# Autodesk Inventor assembly: WheelAssembly3.0
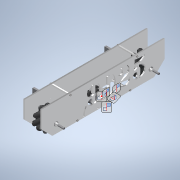
[picture p0: Inventor's stored thumbnail of the model, 180x180]
Saved by Autodesk Inventor 2021 (Build 250183000, 183)
## iProperties
Created: 2017-07-22
Part Number: WheelAssembly3.0
Document SubType Name: Assembly
Designer: User
Mass: 2301.48 g
Surface Area: 4071.67 cm^2
Volume: 902.346 cm^3
Density: 2.55055 g/cm^3
Author: User
## Documents named in this file (22)
- D:\robotics\CAD\2020-21-CAD\Drivetrain\drive train left.iam
- D:\robotics\CAD\COTSParts\Actobotics\535 parts\535198Bearing.25ID.5OD.ipt
- D:\robotics\CAD\COTSParts\Actobotics\Collar.ipt
- D:\robotics\CAD\COTSParts\Fasteners\6-32 SHCS x500.ipt
- D:\robotics\CAD\COTSParts\Fasteners\Hex Standoff 6-32 x2250.ipt
- D:\robotics\CAD\COTSParts\Motors\am-3102NeveRest20 (1)_MIR.ipt
- D:\robotics\CAD\COTSParts\Rev\REV-41-1657MecanumWheelRight.iam
- D:\robotics\CAD\2020-21-CAD\Drivetrain\motor mount.ipt
- D:\robotics\CAD\COTSParts\Tetrix\Tetrix hub - motor.ipt
- D:\robotics\CAD\COTSParts\Actobotics\535 parts\535198Bearing.25ID.5OD_MIR1.ipt
- D:\robotics\CAD\COTSParts\Actobotics\Collar_MIR1.ipt
- D:\robotics\CAD\COTSParts\Rev\REV-41-1657MecanumWheelRight_MIR.iam
- D:\robotics\CAD\2020-21-CAD\Drivetrain\motor mount_MIR.ipt
- D:\robotics\CAD\COTSParts\Motors\am-3102NeveRest20 (1)_MIR_MIR.ipt
- D:\robotics\CAD\COTSParts\andymark\am-3902 am-3903 2in Omni 14mm Hex.ipt
- D:\robotics\CAD\COTSParts\Rev\REV-11-1271.STEP encoders.ipt
- D:\robotics\CAD\COTSParts\Actobotics\637 parts\637222 beval gear\615456 13tooth beval gear.ipt
- D:\robotics\CAD\COTSParts\Actobotics\637 parts\637222 beval gear\615460 26 tooth beval gear.ipt
- D:\robotics\CAD\COTSParts\Tetrix\Tetrix Hub - axle.ipt
- D:\robotics\CAD\2020-21-CAD\Drivetrain\InvertedDrivePlateInsideleft.ipt
- D:\robotics\CAD\2020-21-CAD\custom parts\.25 axle 4.5in.ipt
- D:\robotics\CAD\2020-21-CAD\Drivetrain\InvertedDrivePlateOutsiderleft.ipt
## Components (38 placed, 21 different names)
1. 535198Bearing.25ID.5OD:1 — Insert:86, Mate:157, Mate:158
2. Collar:1 — Insert:86
3. 6-32 SHCS x500:22 — Mate:155, Mate:156
4. 6-32 SHCS x500:23 — Mate:153, Mate:154
5. 6-32 SHCS x500:24 — Mate:139, Mate:140
6. 6-32 SHCS x500:25 — Mate:141, Mate:144
7. REV-41-1657MecanumWheelRight:1 [sub-assembly] — Mate:70, Mate:71, Mate:72, Flush:14
8. motor mount:1 — Mate:66, Mate:67, Mate:113, Mate:168, Mate:169, Mate:170
9. am-3102NeveRest20 (1)_MIR:2 — Mate:66, Mate:67, Angle:2, Mate:112
10. Tetrix hub - motor:1 — Mate:70, Mate:71, Mate:72, Mate:147
11. 535198Bearing.25ID.5OD_MIR1:1 — Insert:151, Mate:145, Mate:146
12. Collar_MIR1:1 — Insert:151
13. 535198Bearing.25ID.5OD_MIR1:2 — Mate:135, Mate:136
14. REV-41-1657MecanumWheelRight_MIR:1 [sub-assembly] — Flush:14, Mate:134, Mate:148
15. motor mount_MIR:1 — Mate:164, Mate:165, Mate:166, Mate:167, Mate:171, Mate:172, Angle:5, Mate:173
16. am-3102NeveRest20 (1)_MIR_MIR:1 — Angle:2, Mate:96, Mate:171, Mate:172, Angle:5, Mate:174
17. am-3902 am-3903 2in Omni 14mm Hex:1 — Mate:89, Mate:90
18. REV-11-1271.STEP encoders:1 — Mate:89, Mate:90, Mate:130, Mate:131, Angle:4
19. 615456 13tooth beval gear:1 — Mate:132, Mate:133
20. 615460 26 tooth beval gear:1 — Mate:93, Mate:94, Mate:96
21. Tetrix Hub - axle:1 — Mate:93, Mate:94
22. 615456 13tooth beval gear:2 — Mate:159, Mate:160
23. 615460 26 tooth beval gear:2 — Mate:174
24. Tetrix Hub - axle:2 — Mate:173
25. 615460 26 tooth beval gear:3 — Mate:113
26. Tetrix Hub - axle:3 — Mate:112
27. InvertedDrivePlateInsideleft:1 — Mate:114, Mate:115, Mate:116, Mate:117, Mate:118, Mate:119, Mate:121, Mate:122, Mate:123, Mate:124, Mate:133, Mate:136, Mate:137, Mate:138, Mate:139, Mate:140, Mate:141, Mate:142, Mate:143, Mate:144, Mate:148, Mate:159, Mate:164, Mate:165, Mate:166, Mate:167, Mate:168, Mate:169, Mate:170
28. 6-32 SHCS x500:27 — Mate:151, Mate:152
29. 6-32 SHCS x500:28 — Mate:149, Mate:150
30. 6-32 SHCS x500:29 — Mate:137, Mate:138
31. 6-32 SHCS x500:30 — Mate:142, Mate:143
32. Hex Standoff 6-32 x2250:3 — Mate:118, Mate:119
33. Hex Standoff 6-32 x2250:4 — Mate:114, Mate:115, Mate:127
34. Hex Standoff 6-32 x2250:5 — Mate:116, Mate:117, Mate:126
35. Hex Standoff 6-32 x2250:6 — Mate:121, Mate:122, Mate:125
36. .25 axle size template:1 — Mate:123, Mate:129, Mate:132, Mate:134, Mate:135
37. .25 axle size template:2 — Mate:124, Mate:128, Mate:147, Mate:157, Mate:160
38. InvertedDrivePlateOutsiderleft:1 — Mate:125, Mate:126, Mate:127, Mate:128, Mate:129, Mate:130, Mate:131, Angle:4, Mate:145, Mate:146, Mate:149, Mate:150, Mate:151, Mate:152, Mate:153, Mate:154, Mate:155, Mate:156, Mate:158
## Relationships (79: Mate 73, Angle 3, Insert 2, Flush 1)
- Insert:86: 535198Bearing.25ID.5OD:1 ↔ Collar:1
- Mate:66: motor mount:1 ↔ am-3102NeveRest20 (1)_MIR:2
- Mate:67: motor mount:1 ↔ am-3102NeveRest20 (1)_MIR:2
- Mate:70: REV-41-1657MecanumWheelRight:1 ↔ Tetrix hub - motor:1
- Mate:71: REV-41-1657MecanumWheelRight:1 ↔ Tetrix hub - motor:1
- Mate:72: REV-41-1657MecanumWheelRight:1 ↔ Tetrix hub - motor:1
- Insert:151: 535198Bearing.25ID.5OD_MIR1:1 ↔ Collar_MIR1:1
- Angle:2 (0 deg): am-3102NeveRest20 (1)_MIR:2 ↔ am-3102NeveRest20 (1)_MIR_MIR:1
- Flush:14: REV-41-1657MecanumWheelRight:1 ↔ REV-41-1657MecanumWheelRight_MIR:1
- Mate:89: am-3902 am-3903 2in Omni 14mm Hex:1 ↔ REV-11-1271.STEP encoders:1
- Mate:90: am-3902 am-3903 2in Omni 14mm Hex:1 ↔ REV-11-1271.STEP encoders:1
- Mate:93: 615460 26 tooth beval gear:1 ↔ Tetrix Hub - axle:1
- Mate:94: 615460 26 tooth beval gear:1 ↔ Tetrix Hub - axle:1
- Mate:96: am-3102NeveRest20 (1)_MIR_MIR:1 ↔ 615460 26 tooth beval gear:1
- [Mate]: 615460 26 tooth beval gear:2 ↔ Tetrix Hub - axle:2
- [Mate]: 615460 26 tooth beval gear:2 ↔ Tetrix Hub - axle:2
- [Mate]: 615460 26 tooth beval gear:3 ↔ Tetrix Hub - axle:3
- [Mate]: 615460 26 tooth beval gear:3 ↔ Tetrix Hub - axle:3
- Mate:112: am-3102NeveRest20 (1)_MIR:2 ↔ Tetrix Hub - axle:3
- Mate:113 (25.4 mm): motor mount:1 ↔ 615460 26 tooth beval gear:3
- Mate:114: InvertedDrivePlateInsideleft:1 ↔ Hex Standoff 6-32 x2250:4
- Mate:115: InvertedDrivePlateInsideleft:1 ↔ Hex Standoff 6-32 x2250:4
- Mate:116: InvertedDrivePlateInsideleft:1 ↔ Hex Standoff 6-32 x2250:5
- Mate:117: InvertedDrivePlateInsideleft:1 ↔ Hex Standoff 6-32 x2250:5
- Mate:118: InvertedDrivePlateInsideleft:1 ↔ Hex Standoff 6-32 x2250:3
- Mate:119: InvertedDrivePlateInsideleft:1 ↔ Hex Standoff 6-32 x2250:3
- Mate:121: InvertedDrivePlateInsideleft:1 ↔ Hex Standoff 6-32 x2250:6
- Mate:122: InvertedDrivePlateInsideleft:1 ↔ Hex Standoff 6-32 x2250:6
- Mate:123: InvertedDrivePlateInsideleft:1 ↔ .25 axle size template:1
- Mate:124: InvertedDrivePlateInsideleft:1 ↔ .25 axle size template:2
- Mate:125: Hex Standoff 6-32 x2250:6 ↔ InvertedDrivePlateOutsiderleft:1
- Mate:126: Hex Standoff 6-32 x2250:5 ↔ InvertedDrivePlateOutsiderleft:1
- Mate:127: Hex Standoff 6-32 x2250:4 ↔ InvertedDrivePlateOutsiderleft:1
- Mate:128: .25 axle size template:2 ↔ InvertedDrivePlateOutsiderleft:1
- Mate:129: .25 axle size template:1 ↔ InvertedDrivePlateOutsiderleft:1
- Mate:130: REV-11-1271.STEP encoders:1 ↔ InvertedDrivePlateOutsiderleft:1
- Mate:131: REV-11-1271.STEP encoders:1 ↔ InvertedDrivePlateOutsiderleft:1
- Angle:4 (-25 deg): REV-11-1271.STEP encoders:1 ↔ InvertedDrivePlateOutsiderleft:1
- Mate:132: 615456 13tooth beval gear:1 ↔ .25 axle size template:1
- Mate:133: 615456 13tooth beval gear:1 ↔ InvertedDrivePlateInsideleft:1
- Mate:134: REV-41-1657MecanumWheelRight_MIR:1 ↔ .25 axle size template:1
- Mate:135: 535198Bearing.25ID.5OD_MIR1:2 ↔ .25 axle size template:1
- Mate:136: 535198Bearing.25ID.5OD_MIR1:2 ↔ InvertedDrivePlateInsideleft:1
- Mate:137: InvertedDrivePlateInsideleft:1 ↔ 6-32 SHCS x500:29
- Mate:138: InvertedDrivePlateInsideleft:1 ↔ 6-32 SHCS x500:29
- Mate:139: 6-32 SHCS x500:24 ↔ InvertedDrivePlateInsideleft:1
- Mate:140: 6-32 SHCS x500:24 ↔ InvertedDrivePlateInsideleft:1
- Mate:141: 6-32 SHCS x500:25 ↔ InvertedDrivePlateInsideleft:1
- Mate:142: InvertedDrivePlateInsideleft:1 ↔ 6-32 SHCS x500:30
- Mate:143: InvertedDrivePlateInsideleft:1 ↔ 6-32 SHCS x500:30
- Mate:144: 6-32 SHCS x500:25 ↔ InvertedDrivePlateInsideleft:1
- Mate:145: 535198Bearing.25ID.5OD_MIR1:1 ↔ InvertedDrivePlateOutsiderleft:1
- Mate:146: 535198Bearing.25ID.5OD_MIR1:1 ↔ InvertedDrivePlateOutsiderleft:1
- Mate:147: Tetrix hub - motor:1 ↔ .25 axle size template:2
- Mate:148 (25.4 mm): REV-41-1657MecanumWheelRight_MIR:1 ↔ InvertedDrivePlateInsideleft:1
- Mate:149: 6-32 SHCS x500:28 ↔ InvertedDrivePlateOutsiderleft:1
- Mate:150: 6-32 SHCS x500:28 ↔ InvertedDrivePlateOutsiderleft:1
- Mate:151: 6-32 SHCS x500:27 ↔ InvertedDrivePlateOutsiderleft:1
- Mate:152: 6-32 SHCS x500:27 ↔ InvertedDrivePlateOutsiderleft:1
- Mate:153: 6-32 SHCS x500:23 ↔ InvertedDrivePlateOutsiderleft:1
- Mate:154: 6-32 SHCS x500:23 ↔ InvertedDrivePlateOutsiderleft:1
- Mate:155: 6-32 SHCS x500:22 ↔ InvertedDrivePlateOutsiderleft:1
- Mate:156: 6-32 SHCS x500:22 ↔ InvertedDrivePlateOutsiderleft:1
- Mate:157: 535198Bearing.25ID.5OD:1 ↔ .25 axle size template:2
- Mate:158: 535198Bearing.25ID.5OD:1 ↔ InvertedDrivePlateOutsiderleft:1
- Mate:159: 615456 13tooth beval gear:2 ↔ InvertedDrivePlateInsideleft:1
- Mate:160: 615456 13tooth beval gear:2 ↔ .25 axle size template:2
- Mate:164: motor mount_MIR:1 ↔ InvertedDrivePlateInsideleft:1
- Mate:165: motor mount_MIR:1 ↔ InvertedDrivePlateInsideleft:1
- Mate:166: motor mount_MIR:1 ↔ InvertedDrivePlateInsideleft:1
- Mate:167: motor mount_MIR:1 ↔ InvertedDrivePlateInsideleft:1
- Mate:168: motor mount:1 ↔ InvertedDrivePlateInsideleft:1
- Mate:169: motor mount:1 ↔ InvertedDrivePlateInsideleft:1
- Mate:170: motor mount:1 ↔ InvertedDrivePlateInsideleft:1
- Mate:171: motor mount_MIR:1 ↔ am-3102NeveRest20 (1)_MIR_MIR:1
- Mate:172: motor mount_MIR:1 ↔ am-3102NeveRest20 (1)_MIR_MIR:1
- Angle:5 (17 deg): motor mount_MIR:1 ↔ am-3102NeveRest20 (1)_MIR_MIR:1
- Mate:173: motor mount_MIR:1 ↔ Tetrix Hub - axle:2
- Mate:174: am-3102NeveRest20 (1)_MIR_MIR:1 ↔ 615460 26 tooth beval gear:2
## Named parameters: d366_d360 = 0 mm, d367_d361 = 0 mm, d382_d360 = 0 mm, d383_d361 = 0 mm
